# Autodesk Inventor assembly: Lever Arm
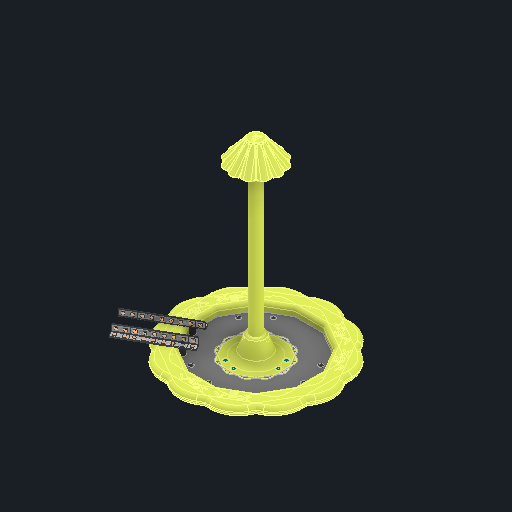
[picture p0: Inventor's stored thumbnail of the model, 512x512]
Saved by Autodesk Inventor 2025 (Build 290162000, 162)
## iProperties
Created: 2024-12-22
Part Number: Lever Arm
Document SubType Name: Assembly
Designer: Averey Ku
Author: Averey Ku
## Documents named in this file (8)
- D:\VEX\High Stakes\CAD\V4\Clamp\Lever Arm.iam
- D:\VEX\High Stakes\V5RC High Stakes Field\276-8868-200.iam
- D:\VEX\High Stakes\CAD\ROBOPROS-CAD-Inventor\Motion\Spacers\Spacer Nylon .375 OD\NSpacer .375 OD x .500.ipt
- D:\VEX\High Stakes\CAD\ROBOPROS-CAD-Inventor\Motion\Spacers\Spacer Nylon .375 OD.ipt
- D:\VEX\High Stakes\CAD\ROBOPROS-CAD-Inventor\Structure\Angle\Aluminum 1x1\Alu Angle 1x1x8.ipt
- D:\VEX\High Stakes\CAD\ROBOPROS-CAD-Inventor\Structure\Angle\Aluminum 1x1\Alu Angle 1x1x7.ipt
- D:\VEX\High Stakes\CAD\ROBOPROS-CAD-Inventor\Structure\Hardware\Screw Steel - Star\SScrew Star Smooth .750.ipt
- D:\VEX\High Stakes\CAD\ROBOPROS-CAD-Inventor\Structure\Hardware\Screw Steel - Star.ipt
## Components (10 placed, 5 different names)
1. 276-8868-200:1 [sub-assembly] — Mate:1, Angle:1, Mate:2, Tangent:1, Tangent:4, Mate:10
2. 276-8868-200:2 [sub-assembly] — Mate:1, Angle:1, Mate:2, Tangent:2, Tangent:3
3. NSpacer .375 OD x .500:1 — Tangent:1, Tangent:2, Mate:8, Insert:7, Insert:8
4. NSpacer .375 OD x .500:2 — Tangent:3, Tangent:4, Mate:9, Insert:9, Insert:10
5. Alu Angle 1x1x8:1 — Mate:5, Insert:6, Mate:7
6. Alu Angle 1x1x8:2 — Mate:5, Insert:5, Mate:6
7. Alu Angle 1x1x7:1 — Insert:5, Mate:6, Mate:9, Insert:9
8. Alu Angle 1x1x7:2 — Insert:6, Mate:7, Mate:8, Mate:10, Insert:7
9. SScrew Star Smooth .750:1 — Insert:8
10. SScrew Star Smooth .750:2 — Insert:10
## Relationships (19: Mate 8, Insert 6, Tangent 4, Angle 1)
- Mate:1: 276-8868-200:1 ↔ 276-8868-200:2
- Angle:1 (30 deg): 276-8868-200:1 ↔ 276-8868-200:2
- Mate:2: 276-8868-200:1 ↔ 276-8868-200:2
- Tangent:1: 276-8868-200:1 ↔ NSpacer .375 OD x .500:1
- Tangent:2: 276-8868-200:2 ↔ NSpacer .375 OD x .500:1
- Tangent:3: 276-8868-200:2 ↔ NSpacer .375 OD x .500:2
- Tangent:4: 276-8868-200:1 ↔ NSpacer .375 OD x .500:2
- Mate:5: Alu Angle 1x1x8:1 ↔ Alu Angle 1x1x8:2
- Insert:5: Alu Angle 1x1x8:2 ↔ Alu Angle 1x1x7:1
- Mate:6: Alu Angle 1x1x8:2 ↔ Alu Angle 1x1x7:1
- Insert:6: Alu Angle 1x1x8:1 ↔ Alu Angle 1x1x7:2
- Mate:7: Alu Angle 1x1x8:1 ↔ Alu Angle 1x1x7:2
- Mate:8: NSpacer .375 OD x .500:1 ↔ Alu Angle 1x1x7:2
- Mate:9: NSpacer .375 OD x .500:2 ↔ Alu Angle 1x1x7:1
- Mate:10: 276-8868-200:1 ↔ Alu Angle 1x1x7:2
- Insert:7: NSpacer .375 OD x .500:1 ↔ Alu Angle 1x1x7:2
- Insert:8: NSpacer .375 OD x .500:1 ↔ SScrew Star Smooth .750:1
- Insert:9: NSpacer .375 OD x .500:2 ↔ Alu Angle 1x1x7:1
- Insert:10: NSpacer .375 OD x .500:2 ↔ SScrew Star Smooth .750:2
